# Autodesk Inventor assembly: testSupportTray
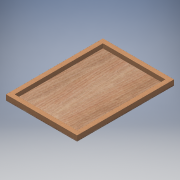
[picture p0: Inventor's stored thumbnail of the model, 180x180]
Saved by Autodesk Inventor 2019 (Build 230136000, 136)
## iProperties
Created: 2019-02-01
Part Number: testSupportTray
Document SubType Name: Assembly
Designer: gaincarlo
Author: gaincarlo
## Documents named in this file (4)
- D:\Giancarlo Bacchio\Documenti\00 - Progetti\30-Inventor\flower vase\testSupportTray.iam
- D:\Giancarlo Bacchio\Documenti\00 - Progetti\30-Inventor\flower vase\testSupport_parts\testBasePlate.ipt
- D:\Giancarlo Bacchio\Documenti\00 - Progetti\30-Inventor\flower vase\testSupport_parts\testsideLong.ipt
- D:\Giancarlo Bacchio\Documenti\00 - Progetti\30-Inventor\flower vase\testSupport_parts\testsideShort.ipt
## Components (5 placed, 3 different names)
1. testBasePlate:1 — Flush:1, Mate:1, Flush:2, Mate:2, Flush:3, Mate:7, Mate:8
2. testsideLong:1 — Flush:2, Mate:2, Mate:3, Flush:7
3. testsideLong:2 — Mate:6, Flush:6, Mate:7, Mate:9
4. testsideShort:1 — Flush:1, Mate:1, Mate:3, Flush:3, Mate:6, Flush:6
5. testsideShort:2 — Mate:8, Mate:9, Flush:7
## Relationships (12: Mate 7, Flush 5)
- Flush:1: testBasePlate:1 ↔ testsideShort:1
- Mate:1: testBasePlate:1 ↔ testsideShort:1
- Flush:2: testBasePlate:1 ↔ testsideLong:1
- Mate:2: testBasePlate:1 ↔ testsideLong:1
- Mate:3: testsideLong:1 ↔ testsideShort:1
- Flush:3: testBasePlate:1 ↔ testsideShort:1
- Mate:6: testsideLong:2 ↔ testsideShort:1
- Flush:6: testsideLong:2 ↔ testsideShort:1
- Mate:7: testBasePlate:1 ↔ testsideLong:2
- Mate:8: testBasePlate:1 ↔ testsideShort:2
- Mate:9: testsideLong:2 ↔ testsideShort:2
- Flush:7: testsideLong:1 ↔ testsideShort:2
